# Autodesk Inventor assembly: mirror_assembly_final
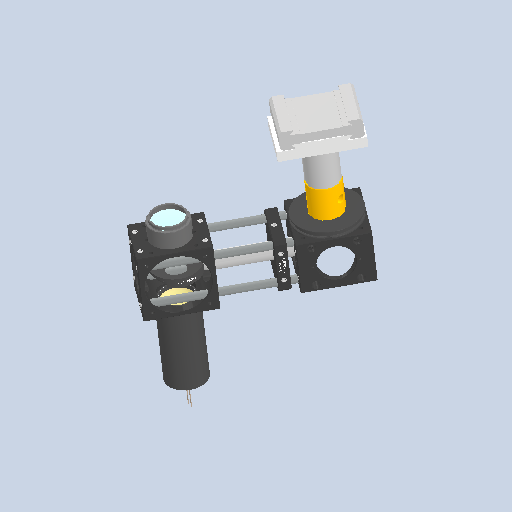
[picture p0: Inventor's stored thumbnail of the model, 512x512]
Saved by Autodesk Inventor 2026.1 (Build 301233000, 233)
## iProperties
Created: 2019-05-24
Part Number: mirror_assembly_final
Document SubType Name: Assembly
Designer: Julian
Author: Julian
## Documents named in this file (11)
- C:\Users\user\Desktop\setup for publishing\LED mount and arm.iam
- C:\Users\user\Desktop\setup for publishing\XT66C2-Step_rail mount.ipt
- C:\Users\user\Desktop\setup for publishing\XT66D2-40-Step_post_mount.ipt
- C:\Users\user\Desktop\setup for publishing\M-PS-1E_1in_70mm_post.ipt
- C:\Users\user\Desktop\setup for publishing\C6WR.ipt
- C:\Users\user\Desktop\setup for publishing\B3C.ipt
- C:\Users\user\Desktop\setup for publishing\ER4.ipt
- C:\Users\user\Desktop\setup for publishing\LED and Diffusor.iam
- C:\Users\user\Desktop\setup for publishing\AC254-075-A.ipt
- C:\Users\user\Desktop\setup for publishing\CP14_M.ipt
- C:\Users\user\Desktop\setup for publishing\ID20_M.ipt
## Components (14 placed, 10 different names)
1. XT66C2-Step_rail mount:1 — Mate:5, Mate:6, Flush:1
2. XT66D2-40-Step_post_mount:1 — Mate:5, Mate:6, Flush:1, Passend:7, Passend:8, Winkel:1
3. M-PS-1E_1in_70mm_post:1 — Passend:7, Passend:8, Passend:11, Passend:12
4. C6WR:1 — Passend:9, Passend:10, Winkel:1, Passend:13, Passend:14, Passend:15, Passend:16, Passend:17, Passend:18, Passend:19, Passend:20, Passend:31
5. C6WR:2 — Passend:21, Passend:22, Fluchtend:2, Passend:23, Passend:24, Passend:25, Passend:26
6. B3C:1 — Passend:9, Passend:10, Passend:11, Passend:12
7. ER4:1 — Passend:14, Passend:17, Passend:21, Fluchtend:2
8. ER4:2 — Passend:16, Passend:19, Passend:22
9. ER4:3 — Passend:15, Passend:20, Passend:30
10. ER4:4 — Passend:13, Passend:18, Passend:29
11. LED and Diffusor:1 [sub-assembly] — Passend:23, Passend:24
12. AC254-075-A:1 — Passend:25, Passend:26
13. CP14_M:1 — Passend:27, Passend:28, Passend:29, Passend:30, Passend:31
14. ID20_M:1 — Passend:27, Passend:28
## Relationships (30: Mate 27, Flush 2, Angle 1)
- Mate:5: XT66C2-Step_rail mount:1 ↔ XT66D2-40-Step_post_mount:1
- Mate:6: XT66C2-Step_rail mount:1 ↔ XT66D2-40-Step_post_mount:1
- Flush:1 (-0.0508 mm): XT66C2-Step_rail mount:1 ↔ XT66D2-40-Step_post_mount:1
- Passend:7 [Mate]: XT66D2-40-Step_post_mount:1 ↔ M-PS-1E_1in_70mm_post:1
- Passend:8 [Mate]: XT66D2-40-Step_post_mount:1 ↔ M-PS-1E_1in_70mm_post:1
- Passend:9 [Mate]: C6WR:1 ↔ B3C:1
- Passend:10 [Mate]: C6WR:1 ↔ B3C:1
- Passend:11 [Mate]: M-PS-1E_1in_70mm_post:1 ↔ B3C:1
- Passend:12 [Mate]: M-PS-1E_1in_70mm_post:1 ↔ B3C:1
- Winkel:1 [Angle] (0 deg): XT66D2-40-Step_post_mount:1 ↔ C6WR:1
- Passend:13 [Mate]: C6WR:1 ↔ ER4:4
- Passend:14 [Mate]: C6WR:1 ↔ ER4:1
- Passend:15 [Mate]: C6WR:1 ↔ ER4:3
- Passend:16 [Mate]: C6WR:1 ↔ ER4:2
- Passend:17 [Mate]: C6WR:1 ↔ ER4:1
- Passend:18 [Mate]: C6WR:1 ↔ ER4:4
- Passend:19 [Mate]: C6WR:1 ↔ ER4:2
- Passend:20 [Mate]: C6WR:1 ↔ ER4:3
- Passend:21 [Mate]: C6WR:2 ↔ ER4:1
- Passend:22 [Mate]: C6WR:2 ↔ ER4:2
- Fluchtend:2 [Flush] (2 mm): C6WR:2 ↔ ER4:1
- Passend:23 [Mate]: C6WR:2 ↔ LED and Diffusor:1
- Passend:24 [Mate]: C6WR:2 ↔ LED and Diffusor:1
- Passend:25 [Mate]: C6WR:2 ↔ AC254-075-A:1
- Passend:26 [Mate]: C6WR:2 ↔ AC254-075-A:1
- Passend:27 [Mate]: CP14_M:1 ↔ ID20_M:1
- Passend:28 [Mate] (-30 mm): CP14_M:1 ↔ ID20_M:1
- Passend:29 [Mate]: ER4:4 ↔ CP14_M:1
- Passend:30 [Mate]: ER4:3 ↔ CP14_M:1
- Passend:31 [Mate] (5 mm): C6WR:1 ↔ CP14_M:1
